# Autodesk Inventor assembly: Assemblyfull one piston
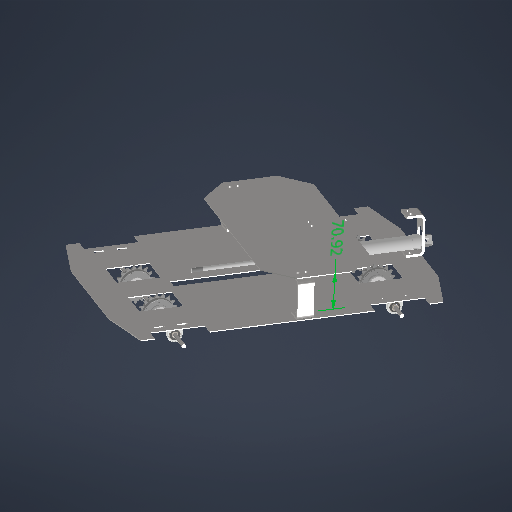
[picture p0: Inventor's stored thumbnail of the model, 512x512]
Saved by Autodesk Inventor 2026.1 (Build 301233020, 233B)
## iProperties
Created: 2026-01-22
Part Number: Assemblyfull one piston
Document SubType Name: Assembly
Designer: user
Author: user
## Documents named in this file (8)
- D:\fall25\machine element design\air vehicle\design new\Assemblyfull one piston.iam
- D:\fall25\machine element design\air vehicle\design new\chassis.ipt
- D:\fall25\machine element design\air vehicle\design new\pillow-block-bearing-p08-1.snapshot.17\Pillow Block P08\Pillow Block P08\Pillow Block P08.ipt
- D:\fall25\machine element design\air vehicle\design new\Assembly shaft 1 sprocect.iam
- D:\fall25\machine element design\air vehicle\design new\piston bracket.ipt
- D:\fall25\machine element design\air vehicle\design new\piston\piston .iam
- D:\fall25\machine element design\air vehicle\design new\chassis up .ipt
- D:\fall25\machine element design\air vehicle\design new\up bracket.ipt
## Components (13 placed, 7 different names)
1. chassis:1 — Mate:1, Mate:2, Mate:3, Mate:4, Mate:5, Mate:6, Mate:7, Mate:8, Mate:9, Mate:10, Mate:11, Mate:12, Mate:15, Mate:16, Mate:17, Mate:18, Mate:19, Mate:20, Mate:23, Mate:24, Mate:25, Mate:26, Mate:27, Mate:28
2. Pillow Block P08:1 — Mate:1, Mate:2, Mate:3, Mate:14
3. Pillow Block P08:2 — Mate:5, Mate:11, Mate:12
4. Pillow Block P08:3 — Mate:6, Mate:7, Mate:8, Mate:13
5. Pillow Block P08:4 — Mate:4, Mate:9, Mate:10
6. Assembly shaft 1 sprocect:1 [sub-assembly] — Mate:13
7. Assembly shaft 1 sprocect:2 [sub-assembly] — Mate:14
8. piston bracket:1 — Mate:15, Mate:19, Mate:20, Mate:22
9. piston bracket:2 — Mate:16, Mate:17, Mate:18, Mate:21
10. piston :1 [sub-assembly] — Mate:21, Mate:22
11. up bracket:1 — Mate:23, Mate:24, Mate:25, Mate:29
12. up bracket:2 — Mate:26, Mate:27, Mate:28, Mate:30, Mate:31
13. chassis up :1 — Mate:29, Mate:30, Mate:31
## Relationships (31: Mate 31)
- Mate:1: chassis:1 ↔ Pillow Block P08:1
- Mate:2: chassis:1 ↔ Pillow Block P08:1
- Mate:3: chassis:1 ↔ Pillow Block P08:1
- Mate:4: chassis:1 ↔ Pillow Block P08:4
- Mate:5: chassis:1 ↔ Pillow Block P08:2
- Mate:6: chassis:1 ↔ Pillow Block P08:3
- Mate:7: chassis:1 ↔ Pillow Block P08:3
- Mate:8: chassis:1 ↔ Pillow Block P08:3
- Mate:9: chassis:1 ↔ Pillow Block P08:4
- Mate:10: chassis:1 ↔ Pillow Block P08:4
- Mate:11: chassis:1 ↔ Pillow Block P08:2
- Mate:12: chassis:1 ↔ Pillow Block P08:2
- Mate:13: Pillow Block P08:3 ↔ Assembly shaft 1 sprocect:1
- Mate:14: Pillow Block P08:1 ↔ Assembly shaft 1 sprocect:2
- Mate:15: chassis:1 ↔ piston bracket:1
- Mate:16: chassis:1 ↔ piston bracket:2
- Mate:17: chassis:1 ↔ piston bracket:2
- Mate:18: chassis:1 ↔ piston bracket:2
- Mate:19: chassis:1 ↔ piston bracket:1
- Mate:20: chassis:1 ↔ piston bracket:1
- Mate:21: piston bracket:2 ↔ piston :1
- Mate:22: piston bracket:1 ↔ piston :1
- Mate:23: chassis:1 ↔ up bracket:1
- Mate:24: chassis:1 ↔ up bracket:1
- Mate:25: chassis:1 ↔ up bracket:1
- Mate:26: chassis:1 ↔ up bracket:2
- Mate:27: chassis:1 ↔ up bracket:2
- Mate:28: chassis:1 ↔ up bracket:2
- Mate:29: up bracket:1 ↔ chassis up :1
- Mate:30: up bracket:2 ↔ chassis up :1
- Mate:31: up bracket:2 ↔ chassis up :1
## Named parameters: sa_0 = 10000
note: some values were not read from the file. Shown as the stored number, unit unknown: "sa_0".
